# Autodesk Inventor assembly: scissor lift
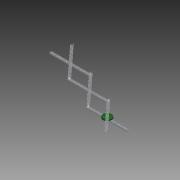
[picture p0: Inventor's stored thumbnail of the model, 180x180]
Saved by Autodesk Inventor 2014 (Build 180170000, 170)
## iProperties
Created: 2014-08-24
Part Number: scissor lift
Document SubType Name: Assembly
Designer: Josef
Author: Josef
## Documents named in this file (4)
- C:\Users\Josef\Documents\Vex parts\#1 sub assemblys\lifts\scissor lift.iam
- C:\Users\Josef\Documents\Vex parts\Metal C-Channels\Aluminum C-Channel 1x2x1x35.ipt
- C:\Users\Josef\Documents\Vex parts\Gears & Pulleys\Imported Components\276-3438\276-3438.ipt
- C:\Users\Josef\Documents\Vex parts\Washers & Spacers\Spacer (Nylon), 0.500''.ipt
## Components (11 placed, 3 different names)
1. Aluminum C-Channel 1x2x1x35:1 — Mate:3, Mate:4, Mate:8, Mate:9
2. Aluminum C-Channel 1x2x1x35:2 — Mate:1, Mate:2, Mate:5, Mate:6, Mate:7
3. 276-3438:1 — Mate:1, Mate:2, Mate:3, Mate:4, Mate:5
4. Spacer (Nylon), 0.500'':1 — Mate:8, Mate:9, Mate:12, Mate:13
5. Spacer (Nylon), 0.500'':2 — Mate:6, Mate:7, Mate:10, Mate:11
6. Aluminum C-Channel 1x2x1x35:3 — Mate:10, Mate:11, Mate:14, Mate:17, Mate:18
7. Aluminum C-Channel 1x2x1x35:4 — Mate:12, Mate:13, Mate:14, Mate:15, Mate:16
8. Aluminum C-Channel 1x2x1x35:5 — Mate:21, Mate:22, Mate:23
9. Aluminum C-Channel 1x2x1x35:6 — Mate:19, Mate:20, Mate:23
10. Spacer (Nylon), 0.500'':3 — Mate:15, Mate:16, Mate:19, Mate:20
11. Spacer (Nylon), 0.500'':4 — Mate:17, Mate:18, Mate:21, Mate:22
## Relationships (23: Mate 23)
- Mate:1: Aluminum C-Channel 1x2x1x35:2 ↔ 276-3438:1
- Mate:2: Aluminum C-Channel 1x2x1x35:2 ↔ 276-3438:1
- Mate:3: Aluminum C-Channel 1x2x1x35:1 ↔ 276-3438:1
- Mate:4: Aluminum C-Channel 1x2x1x35:1 ↔ 276-3438:1
- Mate:5: Aluminum C-Channel 1x2x1x35:2 ↔ 276-3438:1
- Mate:6: Aluminum C-Channel 1x2x1x35:2 ↔ Spacer (Nylon), 0.500'':2
- Mate:7: Aluminum C-Channel 1x2x1x35:2 ↔ Spacer (Nylon), 0.500'':2
- Mate:8: Aluminum C-Channel 1x2x1x35:1 ↔ Spacer (Nylon), 0.500'':1
- Mate:9: Aluminum C-Channel 1x2x1x35:1 ↔ Spacer (Nylon), 0.500'':1
- Mate:10: Spacer (Nylon), 0.500'':2 ↔ Aluminum C-Channel 1x2x1x35:3
- Mate:11: Spacer (Nylon), 0.500'':2 ↔ Aluminum C-Channel 1x2x1x35:3
- Mate:12: Spacer (Nylon), 0.500'':1 ↔ Aluminum C-Channel 1x2x1x35:4
- Mate:13: Spacer (Nylon), 0.500'':1 ↔ Aluminum C-Channel 1x2x1x35:4
- Mate:14: Aluminum C-Channel 1x2x1x35:3 ↔ Aluminum C-Channel 1x2x1x35:4
- Mate:15: Aluminum C-Channel 1x2x1x35:4 ↔ Spacer (Nylon), 0.500'':3
- Mate:16: Aluminum C-Channel 1x2x1x35:4 ↔ Spacer (Nylon), 0.500'':3
- Mate:17: Aluminum C-Channel 1x2x1x35:3 ↔ Spacer (Nylon), 0.500'':4
- Mate:18: Aluminum C-Channel 1x2x1x35:3 ↔ Spacer (Nylon), 0.500'':4
- Mate:19: Aluminum C-Channel 1x2x1x35:6 ↔ Spacer (Nylon), 0.500'':3
- Mate:20: Aluminum C-Channel 1x2x1x35:6 ↔ Spacer (Nylon), 0.500'':3
- Mate:21: Aluminum C-Channel 1x2x1x35:5 ↔ Spacer (Nylon), 0.500'':4
- Mate:22: Aluminum C-Channel 1x2x1x35:5 ↔ Spacer (Nylon), 0.500'':4
- Mate:23: Aluminum C-Channel 1x2x1x35:5 ↔ Aluminum C-Channel 1x2x1x35:6
